# Autodesk Inventor assembly: Ramię z łapką
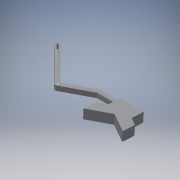
[picture p0: Inventor's stored thumbnail of the model, 180x180]
Saved by Autodesk Inventor 2017 (Build 210142000, 142)
## iProperties
Created: 2018-05-29
Part Number: Ramię z łapką
Document SubType Name: Assembly
Designer: Pies
Author: Pies
## Documents named in this file (3)
- C:\Users\Pies\Desktop\Rzeczy\AGH\Semestr 2\ZIPK\Chwytak\Moj_Chwd_Pytak\Inventorowe chwytaki\Ramię z łapką.iam
- C:\Users\Pies\Desktop\Rzeczy\AGH\Semestr 2\ZIPK\Chwytak\Moj_Chwd_Pytak\Inventorowe chwytaki\Łapka.ipt
- C:\Users\Pies\Desktop\Rzeczy\AGH\Semestr 2\ZIPK\Chwytak\Moj_Chwd_Pytak\Inventorowe chwytaki\Ramię♥.ipt
## Components (2 placed, 2 different names)
1. Łapka:1 — Mate:1, Mate:2
2. Ramię♥:1 — Mate:1, Mate:2
## Relationships (2: Mate 2)
- Mate:1: Łapka:1 ↔ Ramię♥:1
- Mate:2: Łapka:1 ↔ Ramię♥:1
